# Autodesk Inventor assembly: FootCover_MIR
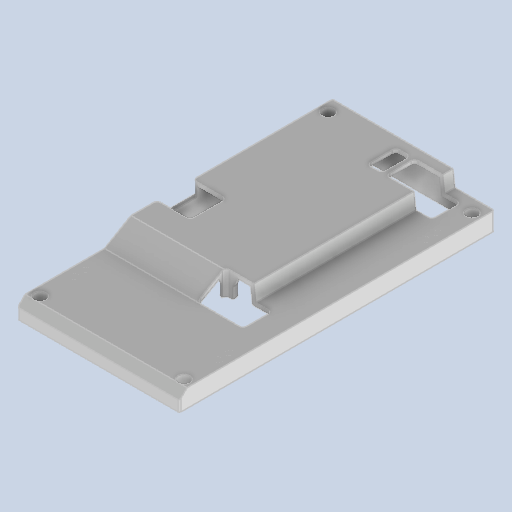
[picture p0: Inventor's stored thumbnail of the model, 512x512]
Saved by Autodesk Inventor 2022.5 (Build 265521000, 521)
## iProperties
Created: 2023-11-25
Part Number: FootCover_MIR
Document SubType Name: Assembly
Designer: Masato Kubotera
Author: Masato Kubotera
## Documents named in this file (2)
- C:\Users\Masato\Documents\Inventor\SUSTAINA-OP\ModelingFiles\LowerBody\Foot\FootCover_MIR.iam
- C:\Users\Masato\Documents\Inventor\SUSTAINA-OP\ModelingFiles\LowerBody\Foot\FootCover_MIR.ipt
## Components (1 placed, 1 different names)
1. FootCover_MIR:1 — Flush:1, Flush:2, Flush:3
## Relationships (3: Flush 3)
- Flush:1: FootCover_MIR:1
- Flush:2: FootCover_MIR:1
- Flush:3: FootCover_MIR:1
